# Autodesk Inventor assembly: HHKS25
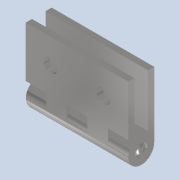
[picture p0: Inventor's stored thumbnail of the model, 180x180]
Saved by Autodesk Inventor 2021.2 (Build 252289000, 289)
## iProperties
Category: PARTsolutions
Company: MISUMI
Part Number: HHKS25
Catalog Web Link: www.cadenas.de
Description: HHKS-Hinges
Vendor: MISUMI
Document SubType Name: Assembly
Designer: partserver
Manufacturer: MISUMI
Mass: 13 g
Surface Area: 26.7538 cm^2
Volume: 1.71963 cm^3
PSOL_IDENT_0: {$CADENAS_DATA\23d-libs\misumi\metric\43_levers_knobs\hhks_assmtab.prj},168 {VTYP=3D},{STYP=ASSTAB},
PSOL_IDENT_1: {NB=HHKS25},{LINA=HHKS25},{NN=HHKS},{DATE=30.10.2020 16:27:20},{GEOMDATE=30.10.2020 15:37:54},{VERSI
PSOL_IDENT_2: ON=},{LINEID=10},{WBVAR=LS},{WBNUMERIC=LS}  {NB=HHKS25},{LINA=HHKS25},{KT=DUMMY},{PN=HHKS25},{TP=HHK
PSOL_IDENT_3: S},{MAT=304 Stainless Steel},{LS=25},{LL=6.0},{L1=13},{L2=0},{L3=0},{NOD=3},{AL=29.4},{WT=13},{PPATH=
PSOL_IDENT_4: assemblies_hhks/hhks_templ.prj}
NB: HHKS25
NN: HHKS
NT: Hinges
NBSYN: $PN.
LINA: HHKS25
CATALOG: Misumi
PN: HHKS25
TP: HHKS
MAT: 304 Stainless Steel
LS: 25
LL: 6
L1: 13
L2: 0
L3: 0
NOD: 3
AL: 29.4
WT: 13
SUPPLIER: MISUMI
ARTICLENO: HHKS25
BOMINFO: HHKS25
CREATOR: CADENAS GmbH
Title: HHKS25
Author: Cadenas PARTsolutions
Comments: Hinges
## Documents named in this file (4)
- C:\Users\Hagihara Yuya\Documents\GrabCAD\NHK2021\BasicParts\よく使う部品（萩原）\Hinge\HHKS25\HHKS25.iam
- C:\Users\Hagihara Yuya\Documents\GrabCAD\NHK2021\BasicParts\よく使う部品（萩原）\Hinge\HHKS25\1HHKS25.ipt
- C:\Users\Hagihara Yuya\Documents\GrabCAD\NHK2021\BasicParts\よく使う部品（萩原）\Hinge\HHKS25\2HHKS25.ipt
- C:\Users\Hagihara Yuya\Documents\GrabCAD\NHK2021\BasicParts\よく使う部品（萩原）\Hinge\HHKS25\pHHKS25.ipt
## Components (3 placed, 3 different names)
1. 1HHKS25:1 — 1_XY@1 <-> 2_XY@2, 1_Z@1 <-> 2_Z@2, 11_XY@1 <-> pin_XY@3, 11_Z@1 <-> pin_Z@3, 11_YZ@1 <-> pin_YZ@3
2. 2HHKS25:1 — 1_XY@1 <-> 2_XY@2, 1_Z@1 <-> 2_Z@2
3. pHHKS25:1 — 11_XY@1 <-> pin_XY@3, 11_Z@1 <-> pin_Z@3, 11_YZ@1 <-> pin_YZ@3
## Relationships (5: Flush 2, Mate 2, Angle 1)
- 1_XY@1 <-> 2_XY@2 [Flush]: 1HHKS25:1 ↔ 2HHKS25:1
- 1_Z@1 <-> 2_Z@2 [Mate]: 1HHKS25:1 ↔ 2HHKS25:1
- 11_XY@1 <-> pin_XY@3 [Flush]: 1HHKS25:1 ↔ pHHKS25:1
- 11_Z@1 <-> pin_Z@3 [Mate]: 1HHKS25:1 ↔ pHHKS25:1
- 11_YZ@1 <-> pin_YZ@3 [Angle] (0 deg): 1HHKS25:1 ↔ pHHKS25:1
